# Autodesk Inventor assembly: bett_sitzbank
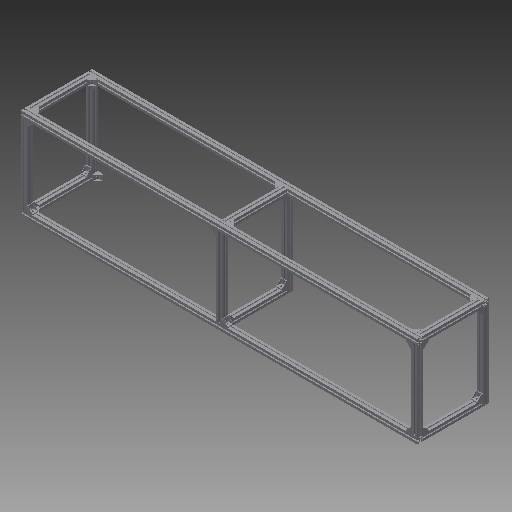
[picture p0: Inventor's stored thumbnail of the model, 512x512]
Saved by Autodesk Inventor 2018 (Build 220112000, 112)
## iProperties
Created: 2020-03-29
Part Number: bett_sitzbank
Material: Generisch
Document SubType Name: Assembly
Designer: wepet
Author: wepet
## Documents named in this file (6)
- C:\Users\wepet\Downloads\anhaenger\current\details\bett\bett_V1_sitzbank.iam
- C:\Users\wepet\Downloads\anhaenger\current\details\bett\details\item_30x30_30cm.ipt
- C:\Users\wepet\Downloads\anhaenger\current\details\bett\details\item_30x30_40cm.ipt
- C:\Users\wepet\Downloads\anhaenger\current\details\bett\details\item_30x30_200cm.ipt
- C:\Users\wepet\Downloads\anhaenger\current\details\bett\details\item_winkel.ipt
- C:\Users\wepet\Downloads\anhaenger\current\details\bett\details\item_30x30_43cm.ipt
## Components (48 placed, 5 different names)
1. item_30x30_30cm:1 — Fluchtend:2, Passend:3, Fluchtend:3, Passend:27
2. item_30x30_40cm:1 — Fluchtend:4, Passend:4, Fluchtend:5, Passend:6, Fluchtend:15, Fluchtend:69, Passend:25, Fluchtend:149, Passend:40
3. item_30x30_200cm:1 — Passend:1, Passend:2, Fluchtend:1, Fluchtend:2, Passend:3, Fluchtend:3, Fluchtend:4, Passend:4, Fluchtend:5, Fluchtend:8, Fluchtend:9, Fluchtend:10, Fluchtend:93, Fluchtend:176, Passend:49, Fluchtend:177, Passend:57, Fluchtend:184, Fluchtend:185, Passend:62
4. item_30x30_200cm:3 — Fluchtend:8, Fluchtend:9, Passend:6, Fluchtend:11, Fluchtend:16, Passend:8, Fluchtend:23, Fluchtend:25, Fluchtend:32, Fluchtend:33, Passend:31, Fluchtend:122, Passend:36
5. item_30x30_200cm:4 — Fluchtend:10, Fluchtend:11, Fluchtend:24, Passend:32, Fluchtend:82, Passend:38, Passend:44, Passend:54, Fluchtend:181, Fluchtend:182, Passend:56
6. item_30x30_43cm:1 — Passend:26, Passend:34, Fluchtend:182, Fluchtend:183, Passend:56, Passend:58, Fluchtend:187, Fluchtend:190, Passend:63, Fluchtend:191
7. item_30x30_30cm:2 — Fluchtend:15, Fluchtend:16, Passend:8, Fluchtend:34, Passend:28, Fluchtend:183
8. item_30x30_30cm:3 — Fluchtend:20, Fluchtend:22, Passend:12, Passend:20, Fluchtend:185, Passend:59, Fluchtend:193
9. item_30x30_40cm:3 — Fluchtend:19, Fluchtend:21, Passend:12, Fluchtend:25, Fluchtend:71, Passend:17, Fluchtend:175, Fluchtend:179, Passend:60
10. item_30x30_43cm:3 — Fluchtend:18, Fluchtend:21, Passend:9, Passend:10, Passend:19, Fluchtend:181, Passend:61, Fluchtend:186, Passend:65
11. item_30x30_30cm:4 — Fluchtend:18, Fluchtend:19, Fluchtend:20, Fluchtend:22, Passend:9, Passend:10, Fluchtend:23, Fluchtend:24, Passend:18, Passend:29
12. item_30x30_30cm:5 — Passend:23, Passend:50, Fluchtend:184
13. item_30x30_40cm:5 — Fluchtend:32, Fluchtend:70, Passend:21, Fluchtend:180, Passend:53
14. item_30x30_43cm:2 — Passend:22, Passend:39, Passend:55, Passend:64, Fluchtend:192
15. item_30x30_30cm:6 — Fluchtend:33, Fluchtend:34, Passend:24, Passend:45, Passend:46
16. item_winkel:5 — Fluchtend:42, Fluchtend:43, Fluchtend:44, Fluchtend:45, Fluchtend:48
17. item_winkel:6 — Fluchtend:42, Fluchtend:47, Fluchtend:48, Passend:23
18. item_winkel:7 — Fluchtend:44, Fluchtend:46, Fluchtend:47, Fluchtend:70, Passend:21
19. item_winkel:8 — Fluchtend:43, Fluchtend:45, Fluchtend:46, Passend:22, Passend:24
20. item_winkel:9 — Fluchtend:71
21. item_winkel:10 — Passend:20
22. item_winkel:11 — Passend:17, Passend:18
23. item_winkel:12 — Passend:19
24. item_winkel:13 — Passend:26, Passend:27
25. item_winkel:14 — Passend:25
26. item_winkel:15 — Fluchtend:69, Passend:28
27. item_winkel:16
28. item_winkel:17 — Passend:32, Passend:45
29. item_winkel:19 — Passend:29, Passend:31, Fluchtend:94
30. item_winkel:20 — Fluchtend:82
31. item_winkel:22 — Fluchtend:177, Passend:50
32. item_winkel:23 — Fluchtend:93, Fluchtend:94, Passend:59
33. item_winkel:25 — Passend:58
34. item_winkel:26 — Fluchtend:122, Passend:34
35. item_winkel:27 — Passend:36, Passend:46
36. item_winkel:30 — Fluchtend:176, Passend:49
37. item_winkel:34 — Fluchtend:187
38. item_winkel:35 — Passend:54, Passend:55
39. item_winkel:37 — Fluchtend:149, Passend:40
40. item_winkel:38 — Passend:38
41. item_winkel:40 — Passend:39, Passend:57
42. item_winkel:43 — Passend:44, Passend:61, Fluchtend:186
43. item_winkel:46 — Fluchtend:180, Passend:53
44. item_winkel:47 — Fluchtend:175
45. item_winkel:48 — Fluchtend:179, Passend:60, Passend:62
46. item_winkel:49 — Fluchtend:189, Passend:65, Fluchtend:193
47. item_winkel:50 — Fluchtend:188, Fluchtend:189, Fluchtend:190, Passend:64, Fluchtend:192
48. item_winkel:51 — Fluchtend:188, Passend:63, Fluchtend:191
## Relationships (160: Flush 110, Mate 50)
- Passend:1 [Mate]: item_30x30_200cm:1
- Passend:2 [Mate]: item_30x30_200cm:1
- Fluchtend:1 [Flush]: item_30x30_200cm:1
- Fluchtend:2 [Flush]: item_30x30_30cm:1 ↔ item_30x30_200cm:1
- Passend:3 [Mate]: item_30x30_30cm:1 ↔ item_30x30_200cm:1
- Fluchtend:3 [Flush]: item_30x30_30cm:1 ↔ item_30x30_200cm:1
- Fluchtend:4 [Flush]: item_30x30_40cm:1 ↔ item_30x30_200cm:1
- Passend:4 [Mate]: item_30x30_40cm:1 ↔ item_30x30_200cm:1
- Fluchtend:5 [Flush]: item_30x30_40cm:1 ↔ item_30x30_200cm:1
- Fluchtend:8 [Flush]: item_30x30_200cm:1 ↔ item_30x30_200cm:3
- Fluchtend:9 [Flush]: item_30x30_200cm:1 ↔ item_30x30_200cm:3
- Passend:6 [Mate]: item_30x30_40cm:1 ↔ item_30x30_200cm:3
- Fluchtend:10 [Flush]: item_30x30_200cm:1 ↔ item_30x30_200cm:4
- Fluchtend:11 [Flush]: item_30x30_200cm:3 ↔ item_30x30_200cm:4
- Fluchtend:15 [Flush]: item_30x30_40cm:1 ↔ item_30x30_30cm:2
- Fluchtend:16 [Flush]: item_30x30_200cm:3 ↔ item_30x30_30cm:2
- Passend:8 [Mate]: item_30x30_200cm:3 ↔ item_30x30_30cm:2
- [Flush]: item_30x30_40cm:3 ↔ item_30x30_30cm:4
- Fluchtend:18 [Flush]: item_30x30_43cm:3 ↔ item_30x30_30cm:4
- Fluchtend:19 [Flush]: item_30x30_40cm:3 ↔ item_30x30_30cm:4
- Fluchtend:20 [Flush]: item_30x30_30cm:3 ↔ item_30x30_30cm:4
- Fluchtend:21 [Flush]: item_30x30_40cm:3 ↔ item_30x30_43cm:3
- Fluchtend:22 [Flush]: item_30x30_30cm:3 ↔ item_30x30_30cm:4
- Passend:9 [Mate]: item_30x30_43cm:3 ↔ item_30x30_30cm:4
- Passend:10 [Mate]: item_30x30_43cm:3 ↔ item_30x30_30cm:4
- Passend:12 [Mate]: item_30x30_30cm:3 ↔ item_30x30_40cm:3
- Fluchtend:23 [Flush]: item_30x30_200cm:3 ↔ item_30x30_30cm:4
- Fluchtend:24 [Flush]: item_30x30_200cm:4 ↔ item_30x30_30cm:4
- Fluchtend:25 [Flush]: item_30x30_200cm:3 ↔ item_30x30_40cm:3
- [Flush]: item_30x30_40cm:5 ↔ item_30x30_30cm:6
- [Flush]: item_30x30_43cm:2 ↔ item_30x30_30cm:6
- [Flush]: item_30x30_40cm:5 ↔ item_30x30_30cm:6
- [Flush]: item_30x30_30cm:5 ↔ item_30x30_30cm:6
- [Flush]: item_30x30_40cm:5 ↔ item_30x30_43cm:2
- [Flush]: item_30x30_30cm:5 ↔ item_30x30_30cm:6
- [Mate]: item_30x30_43cm:2 ↔ item_30x30_30cm:6
- [Mate]: item_30x30_43cm:2 ↔ item_30x30_30cm:6
- [Mate]: item_30x30_30cm:5 ↔ item_30x30_40cm:5
- Fluchtend:32 [Flush]: item_30x30_200cm:3 ↔ item_30x30_40cm:5
- Fluchtend:33 [Flush]: item_30x30_200cm:3 ↔ item_30x30_30cm:6
- Fluchtend:34 [Flush] (98.5 mm): item_30x30_30cm:2 ↔ item_30x30_30cm:6
- [Flush]: item_winkel:5 ↔ item_winkel:8
- [Flush]: item_winkel:5 ↔ item_winkel:7
- [Flush]: item_winkel:5 ↔ item_winkel:6
- Fluchtend:42 [Flush]: item_winkel:5 ↔ item_winkel:6
- Fluchtend:43 [Flush]: item_winkel:5 ↔ item_winkel:8
- Fluchtend:44 [Flush]: item_winkel:5 ↔ item_winkel:7
- Fluchtend:45 [Flush]: item_winkel:5 ↔ item_winkel:8
- Fluchtend:46 [Flush]: item_winkel:7 ↔ item_winkel:8
- Fluchtend:47 [Flush]: item_winkel:6 ↔ item_winkel:7
- Fluchtend:48 [Flush]: item_winkel:5 ↔ item_winkel:6
- [Flush]: item_winkel:9 ↔ item_winkel:12
- [Flush]: item_winkel:9 ↔ item_winkel:11
- [Flush]: item_winkel:9 ↔ item_winkel:10
- [Flush]: item_winkel:9 ↔ item_winkel:10
- [Flush]: item_winkel:9 ↔ item_winkel:12
- [Flush]: item_winkel:9 ↔ item_winkel:11
- [Flush]: item_winkel:9 ↔ item_winkel:12
- [Flush]: item_winkel:11 ↔ item_winkel:12
- [Flush]: item_winkel:10 ↔ item_winkel:11
- [Flush]: item_winkel:9 ↔ item_winkel:10
- [Flush]: item_winkel:13 ↔ item_winkel:16
- [Flush]: item_winkel:13 ↔ item_winkel:15
- [Flush]: item_winkel:13 ↔ item_winkel:14
- [Flush]: item_winkel:13 ↔ item_winkel:14
- [Flush]: item_winkel:13 ↔ item_winkel:16
- [Flush]: item_winkel:13 ↔ item_winkel:15
- [Flush]: item_winkel:13 ↔ item_winkel:16
- [Flush]: item_winkel:15 ↔ item_winkel:16
- [Flush]: item_winkel:14 ↔ item_winkel:15
- [Flush]: item_winkel:13 ↔ item_winkel:14
- Fluchtend:69 [Flush]: item_30x30_40cm:1 ↔ item_winkel:15
- Fluchtend:70 [Flush]: item_30x30_40cm:5 ↔ item_winkel:7
- Fluchtend:71 [Flush]: item_30x30_40cm:3 ↔ item_winkel:9
- Passend:17 [Mate]: item_30x30_40cm:3 ↔ item_winkel:11
- Passend:18 [Mate]: item_30x30_30cm:4 ↔ item_winkel:11
- Passend:19 [Mate]: item_30x30_43cm:3 ↔ item_winkel:12
- Passend:20 [Mate]: item_30x30_30cm:3 ↔ item_winkel:10
- Passend:21 [Mate]: item_30x30_40cm:5 ↔ item_winkel:7
- Passend:22 [Mate]: item_30x30_43cm:2 ↔ item_winkel:8
- Passend:23 [Mate]: item_30x30_30cm:5 ↔ item_winkel:6
- Passend:24 [Mate]: item_30x30_30cm:6 ↔ item_winkel:8
- Passend:25 [Mate]: item_30x30_40cm:1 ↔ item_winkel:14
- Passend:26 [Mate]: item_30x30_43cm:1 ↔ item_winkel:13
- Passend:27 [Mate]: item_30x30_30cm:1 ↔ item_winkel:13
- Passend:28 [Mate]: item_30x30_30cm:2 ↔ item_winkel:15
- [Flush]: item_winkel:17 ↔ item_winkel:20
- [Flush]: item_winkel:17 ↔ item_winkel:19
- [Flush]: item_winkel:17 ↔ item_winkel:20
- [Flush]: item_winkel:17 ↔ item_winkel:19
- [Flush]: item_winkel:17 ↔ item_winkel:20
- [Flush]: item_winkel:19 ↔ item_winkel:20
- Passend:29 [Mate]: item_30x30_30cm:4 ↔ item_winkel:19
- Passend:31 [Mate]: item_30x30_200cm:3 ↔ item_winkel:19
- Passend:32 [Mate]: item_30x30_200cm:4 ↔ item_winkel:17
- Fluchtend:82 [Flush]: item_30x30_200cm:4 ↔ item_winkel:20
- [Flush]: item_winkel:22 ↔ item_winkel:23
- Fluchtend:93 [Flush]: item_30x30_200cm:1 ↔ item_winkel:23
- Fluchtend:94 [Flush]: item_winkel:19 ↔ item_winkel:23
- [Flush]: item_winkel:25 ↔ item_winkel:27
- [Flush]: item_winkel:25 ↔ item_winkel:26
- [Flush]: item_winkel:25 ↔ item_winkel:26
- [Flush]: item_winkel:25 ↔ item_winkel:27
- [Flush]: item_winkel:26 ↔ item_winkel:27
- [Flush]: item_winkel:25 ↔ item_winkel:26
- [Flush]: item_winkel:26 ↔ item_winkel:30
- Fluchtend:122 [Flush]: item_30x30_200cm:3 ↔ item_winkel:26
- Passend:34 [Mate]: item_30x30_43cm:1 ↔ item_winkel:26
- Passend:36 [Mate]: item_30x30_200cm:3 ↔ item_winkel:27
- [Flush]: item_winkel:34 ↔ item_winkel:35
- [Flush]: item_winkel:37 ↔ item_winkel:40
- [Flush]: item_winkel:37 ↔ item_winkel:38
- [Flush]: item_winkel:37 ↔ item_winkel:38
- [Flush]: item_winkel:37 ↔ item_winkel:40
- [Flush]: item_winkel:37 ↔ item_winkel:40
- [Flush]: item_winkel:37 ↔ item_winkel:38
- [Flush]: item_winkel:34 ↔ item_winkel:38
- Passend:38 [Mate]: item_30x30_200cm:4 ↔ item_winkel:38
- Passend:39 [Mate]: item_30x30_43cm:2 ↔ item_winkel:40
- Fluchtend:149 [Flush]: item_30x30_40cm:1 ↔ item_winkel:37
- Passend:40 [Mate]: item_30x30_40cm:1 ↔ item_winkel:37
- [Flush]: item_winkel:47 ↔ item_winkel:48
- [Flush]: item_winkel:46 ↔ item_winkel:47
- [Flush]: item_winkel:43 ↔ item_winkel:47
- Passend:44 [Mate]: item_30x30_200cm:4 ↔ item_winkel:43
- Fluchtend:175 [Flush]: item_30x30_40cm:3 ↔ item_winkel:47
- Passend:45 [Mate]: item_30x30_30cm:6 ↔ item_winkel:17
- Passend:46 [Mate]: item_30x30_30cm:6 ↔ item_winkel:27
- Fluchtend:176 [Flush]: item_30x30_200cm:1 ↔ item_winkel:30
- Passend:49 [Mate]: item_30x30_200cm:1 ↔ item_winkel:30
- Fluchtend:177 [Flush]: item_30x30_200cm:1 ↔ item_winkel:22
- Passend:50 [Mate]: item_30x30_30cm:5 ↔ item_winkel:22
- Fluchtend:179 [Flush]: item_30x30_40cm:3 ↔ item_winkel:48
- Fluchtend:180 [Flush]: item_30x30_40cm:5 ↔ item_winkel:46
- Passend:53 [Mate]: item_30x30_40cm:5 ↔ item_winkel:46
- Passend:54 [Mate]: item_30x30_200cm:4 ↔ item_winkel:35
- Passend:55 [Mate]: item_30x30_43cm:2 ↔ item_winkel:35
- Fluchtend:181 [Flush]: item_30x30_200cm:4 ↔ item_30x30_43cm:3
- Fluchtend:182 [Flush]: item_30x30_200cm:4 ↔ item_30x30_43cm:1
- Fluchtend:183 [Flush]: item_30x30_43cm:1 ↔ item_30x30_30cm:2
- Passend:56 [Mate]: item_30x30_200cm:4 ↔ item_30x30_43cm:1
- Passend:57 [Mate]: item_30x30_200cm:1 ↔ item_winkel:40
- Passend:58 [Mate]: item_30x30_43cm:1 ↔ item_winkel:25
- Fluchtend:184 [Flush]: item_30x30_200cm:1 ↔ item_30x30_30cm:5
- Fluchtend:185 [Flush]: item_30x30_200cm:1 ↔ item_30x30_30cm:3
- Passend:59 [Mate]: item_30x30_30cm:3 ↔ item_winkel:23
- Passend:60 [Mate]: item_30x30_40cm:3 ↔ item_winkel:48
- Passend:61 [Mate]: item_30x30_43cm:3 ↔ item_winkel:43
- Fluchtend:186 [Flush]: item_30x30_43cm:3 ↔ item_winkel:43
- Passend:62 [Mate]: item_30x30_200cm:1 ↔ item_winkel:48
- Fluchtend:187 [Flush]: item_30x30_43cm:1 ↔ item_winkel:34
- Fluchtend:188 [Flush]: item_winkel:50 ↔ item_winkel:51
- Fluchtend:189 [Flush]: item_winkel:49 ↔ item_winkel:50
- Fluchtend:190 [Flush]: item_30x30_43cm:1 ↔ item_winkel:50
- Passend:63 [Mate]: item_30x30_43cm:1 ↔ item_winkel:51
- Fluchtend:191 [Flush]: item_30x30_43cm:1 ↔ item_winkel:51
- Passend:64 [Mate]: item_30x30_43cm:2 ↔ item_winkel:50
- Fluchtend:192 [Flush]: item_30x30_43cm:2 ↔ item_winkel:50
- Passend:65 [Mate]: item_30x30_43cm:3 ↔ item_winkel:49
- Fluchtend:193 [Flush]: item_30x30_30cm:3 ↔ item_winkel:49
## Named parameters: d24_d21 = 0 mm, d37_d26 = 0 mm, d38_d27 = 0 mm, d39_d28 = 0 mm, d40_d29 = 0 mm, d41_d30 = 0 mm, d42_d31 = 0 mm, d44_d33 = 0 mm, d45_d24_d21 = 0 mm, d46_d25 = 0 mm, d61_d60 = 0 mm, d62_d58 = 0 mm, d63_d59 = 0 mm, d71_d61_d60 = 0 mm, d72_d62_d58 = 0 mm, d73_d63_d59 = 0 mm, d74_d64 = 0 mm, d75_d65 = 0 mm, d76_d66 = 0 mm, d77_d67 = 0 mm, d78_d68 = 0 mm, d79_d69 = 0 mm, d80_d70 = 0 mm, d81_d61_d60 = 0 mm, d82_d62_d58 = 0 mm, d83_d63_d59 = 0 mm, d84_d64 = 0 mm, d85_d65 = 0 mm, d86_d66 = 0 mm, d87_d67 = 0 mm, d88_d68 = 0 mm, d89_d69 = 0 mm, d90_d70 = 0 mm, d107_d62_d58 = 0 mm, d108_d63_d59 = 0 mm, d110_d65 = 0 mm, d111_d66 = 0 mm, d112_d67 = 0 mm, d113_d68 = 0 mm, d129_d114_d69 = 0 mm, d136_d106_d61_d60 = 0 mm, d138_d108_d63_d59 = 0 mm, d139_d109_d64 = 0 mm, d141_d111_d66 = 0 mm, d144_d114_d69 = 0 mm, d145_d115_d70 = 0 mm, d157_d133 = 0 mm, d174_d114_d69 = 0 mm, d176_d121_d106_d61_d60 = 0 mm, d177_d122_d107_d62_d58 = 0 mm, d179_d124_d109_d64 = 0 mm, d180_d125_d110_d65 = 0 mm, d182_d127_d112_d67 = 0 mm, d185_d130_d115_d70 = 0 mm, d187_d133 = 0 mm, d213_d183_d128_d113_d68 = 0 mm, d214_d184_d129_d114_d69 = 0 mm, d216_d186_d132 = 0 mm
